# Autodesk Inventor assembly: BodyAssembly
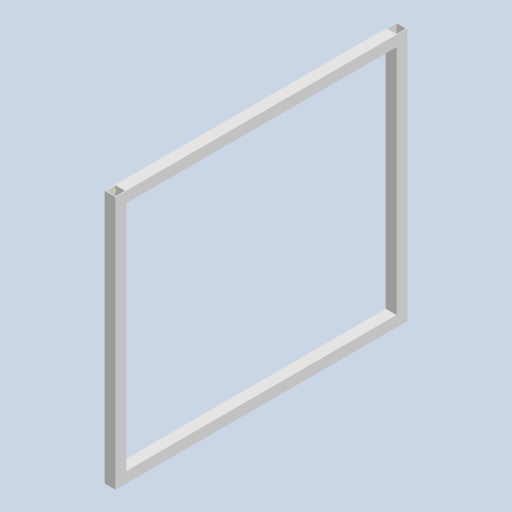
[picture p0: Inventor's stored thumbnail of the model, 512x512]
Saved by Autodesk Inventor 2023 (Build 270158000, 158)
## iProperties
Created: 2023-09-27
Part Number: BodyAssembly
Document SubType Name: Assembly
Designer: Megan
Author: Megan
## Documents named in this file (3)
- C:\Users\megan\OneDrive\Documents\GitHub\BehrendURCMechanical\CAD\Chassis V3\BodyAssembly.iam
- C:\Users\megan\OneDrive\Documents\GitHub\BehrendURCMechanical\CAD\Chassis V3\60cmTube.ipt
- C:\Users\megan\OneDrive\Documents\GitHub\BehrendURCMechanical\CAD\Chassis V3\64cmTube.ipt
## Components (4 placed, 2 different names)
1. 60cmTube:1 — Mate:1, Flush:1, Flush:2, Mate:2, Flush:3, Flush:4
2. 60cmTube:2 — Mate:3, Flush:5, Flush:6
3. 64cmTube:1 — Mate:1, Flush:1, Flush:2, Mate:3, Flush:5, Flush:6
4. 64cmTube:2 — Mate:2, Flush:3, Flush:4
## Relationships (9: Flush 6, Mate 3)
- Mate:1: 60cmTube:1 ↔ 64cmTube:1
- Flush:1: 60cmTube:1 ↔ 64cmTube:1
- Flush:2: 60cmTube:1 ↔ 64cmTube:1
- Mate:2: 60cmTube:1 ↔ 64cmTube:2
- Flush:3: 60cmTube:1 ↔ 64cmTube:2
- Flush:4: 60cmTube:1 ↔ 64cmTube:2
- Mate:3: 60cmTube:2 ↔ 64cmTube:1
- Flush:5: 60cmTube:2 ↔ 64cmTube:1
- Flush:6: 60cmTube:2 ↔ 64cmTube:1
